# Autodesk Inventor assembly: Сборка1
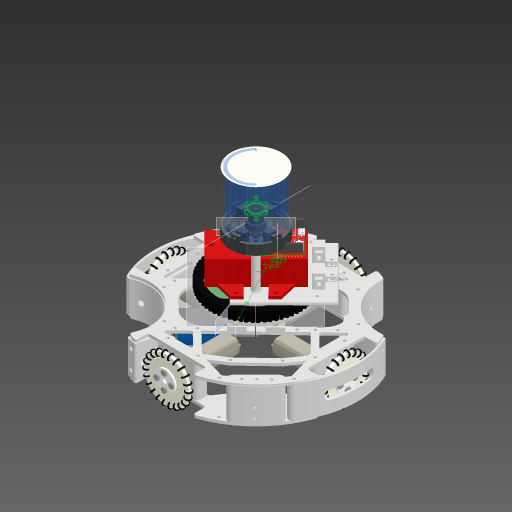
[picture p0: Inventor's stored thumbnail of the model, 512x512]
Saved by Autodesk Inventor 2023 (Build 270158000, 158)
## iProperties
Created: 2025-09-24
Part Number: Сборка1
Document SubType Name: Assembly
Designer: daa
Author: daa
## Documents named in this file (3)
- C:\Users\daa\Documents\DASH_V2\omni_platforma\Сборка1.iam
- C:\Users\daa\Documents\DASH_V2\omni_platforma\omni_platformav222.iam
- C:\Users\daa\Documents\DASH_V2\tower_V2.iam
## Components (2 placed, 2 different names)
1. omni_platformav222:1 [sub-assembly] — Совмещение:1
2. tower_V2:1 [sub-assembly] — Совмещение:1
## Relationships (1: Mate 1)
- Совмещение:1 [Mate]: omni_platformav222:1 ↔ tower_V2:1
